# Autodesk Inventor assembly: Full_Design
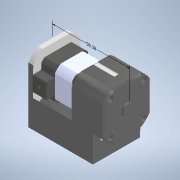
[picture p0: Inventor's stored thumbnail of the model, 180x180]
Saved by Autodesk Inventor 2022 (Build 260153000, 153)
## iProperties
Created: 2022-02-10
Part Number: Full_Design
Document SubType Name: Assembly
Designer: Mlees
Author: Mlees
## Documents named in this file (12)
- C:\Users\Mlees\Desktop\504Engineering\Stepper-Servo_Based_Robotic_Arm\Designs\Version_7\Full_Design.iam
- C:\Users\Mlees\Desktop\504Engineering\Stepper-Servo_Based_Robotic_Arm\Designs\Version_7\Downloaded_Parts\124125202-9-stp-mtr-17040w\stp-mtr-17040w.ipt
- C:\Users\Mlees\Desktop\504Engineering\Stepper-Servo_Based_Robotic_Arm\Designs\Version_7\Created_Parts\Combined_Gear_Box.ipt
- C:\Users\Mlees\Desktop\504Engineering\Stepper-Servo_Based_Robotic_Arm\Designs\Version_7\Created_Parts\Combined_Gear_Box_Modified.ipt
- C:\Users\Mlees\Desktop\504Engineering\Stepper-Servo_Based_Robotic_Arm\Designs\Version_7\Downloaded_Parts\nema17-speed-reducer-1.snapshot.9\M3 Insert 5D x 6L.step.ipt
- C:\Users\Mlees\Desktop\504Engineering\Stepper-Servo_Based_Robotic_Arm\Designs\Version_7\Downloaded_Parts\91290A101_Black-Oxide Alloy Steel Socket Head Screw_M3_6mm.ipt
- C:\Users\Mlees\Desktop\504Engineering\Stepper-Servo_Based_Robotic_Arm\Designs\Version_7\Downloaded_Parts\91290A059_Black-Oxide Alloy Steel Socket Head Screw_M3_30mm.ipt
- C:\Users\Mlees\Desktop\504Engineering\Stepper-Servo_Based_Robotic_Arm\Designs\Version_7\Created_Parts\24_Teeth_Sun_Gear.ipt
- C:\Users\Mlees\Desktop\504Engineering\Stepper-Servo_Based_Robotic_Arm\Designs\Version_7\Created_Parts\Planet_Carrier_Modifed_with_sun_gear.ipt
- C:\Users\Mlees\Desktop\504Engineering\Stepper-Servo_Based_Robotic_Arm\Designs\Version_7\Created_Parts\36_Teeth_Planet_Gear.ipt
- C:\Users\Mlees\Desktop\504Engineering\Stepper-Servo_Based_Robotic_Arm\Designs\Version_7\Created_Parts\Plamet_Carrier.ipt
- C:\Users\Mlees\Desktop\504Engineering\Stepper-Servo_Based_Robotic_Arm\Designs\Version_7\Created_Parts\Gear_Cover_modified.ipt
## Components (29 placed, 11 different names)
1. Combined_Gear_Box:1 — Rigid:1, Rigid:2, Rigid:3, Rigid:4, Rigid:7, Rigid:8, Rotational:1, Rotational:2, Rotational:3, Rotational:4, Rotational:5, Rotational:6, Rigid:9
2. Combined_Gear_Box_Modified:1 — Rigid:5, Rigid:6, Rigid:7
3. M3 Insert 5D x 6L.step:1 — Rigid:2
4. M3 Insert 5D x 6L.step:2 — Rigid:1
5. M3 Insert 5D x 6L.step:3 — Rigid:3
6. M3 Insert 5D x 6L.step:4 — Rigid:4
7. M3 Insert 5D x 6L.step:5 — Rigid:6
8. M3 Insert 5D x 6L.step:6 — Rigid:5
9. stp-mtr-17040w:1 — Rigid:8, Rotational:7, Rotational:11
10. 91290A101_Black-Oxide Alloy Steel Socket Head Screw_M3_6mm:1 — Rotational:1
11. 91290A101_Black-Oxide Alloy Steel Socket Head Screw_M3_6mm:2 — Rotational:2
12. 91290A101_Black-Oxide Alloy Steel Socket Head Screw_M3_6mm:3 — Rotational:3
13. 91290A101_Black-Oxide Alloy Steel Socket Head Screw_M3_6mm:4 — Rotational:4
14. 91290A059_Black-Oxide Alloy Steel Socket Head Screw_M3_30mm:1 — Rotational:6
15. 91290A059_Black-Oxide Alloy Steel Socket Head Screw_M3_30mm:2 — Rotational:5
16. 24_Teeth_Sun_Gear:1 — Rotational:7
17. Planet_Carrier_Modifed_with_sun_gear:1 — Rotational:8, Rotational:9, Rotational:10, Rotational:11, Rotational:15
18. 36_Teeth_Planet_Gear:1 — Rotational:9
19. 36_Teeth_Planet_Gear:2 — Rotational:8
20. 36_Teeth_Planet_Gear:3 — Rotational:10
21. 36_Teeth_Planet_Gear:4 — Rotational:12
22. 36_Teeth_Planet_Gear:5 — Rotational:13
23. 36_Teeth_Planet_Gear:6 — Rotational:14
24. Plamet_Carrier:1 — Rotational:12, Rotational:13, Rotational:14, Rotational:15
25. Gear_Cover_modified:1 — Rigid:9, Rotational:16, Rotational:17, Rotational:18, Rotational:19
26. 91290A059_Black-Oxide Alloy Steel Socket Head Screw_M3_30mm:3 — Rotational:16
27. 91290A059_Black-Oxide Alloy Steel Socket Head Screw_M3_30mm:4 — Rotational:17
28. 91290A059_Black-Oxide Alloy Steel Socket Head Screw_M3_30mm:5 — Rotational:18
29. 91290A059_Black-Oxide Alloy Steel Socket Head Screw_M3_30mm:6 — Rotational:19
## Relationships (28: RevoluteJoint 19, WeldJoint 9)
- Rigid:1 [WeldJoint]: Combined_Gear_Box:1 ↔ M3 Insert 5D x 6L.step:2
- Rigid:2 [WeldJoint]: Combined_Gear_Box:1 ↔ M3 Insert 5D x 6L.step:1
- Rigid:3 [WeldJoint]: Combined_Gear_Box:1 ↔ M3 Insert 5D x 6L.step:3
- Rigid:4 [WeldJoint]: Combined_Gear_Box:1 ↔ M3 Insert 5D x 6L.step:4
- Rigid:5 [WeldJoint]: Combined_Gear_Box_Modified:1 ↔ M3 Insert 5D x 6L.step:6
- Rigid:6 [WeldJoint]: Combined_Gear_Box_Modified:1 ↔ M3 Insert 5D x 6L.step:5
- Rigid:7 [WeldJoint]: Combined_Gear_Box:1 ↔ Combined_Gear_Box_Modified:1
- Rigid:8 [WeldJoint]: Combined_Gear_Box:1 ↔ stp-mtr-17040w:1
- Rotational:1 [RevoluteJoint]: Combined_Gear_Box:1 ↔ 91290A101_Black-Oxide Alloy Steel Socket Head Screw_M3_6mm:1
- Rotational:2 [RevoluteJoint]: Combined_Gear_Box:1 ↔ 91290A101_Black-Oxide Alloy Steel Socket Head Screw_M3_6mm:2
- Rotational:3 [RevoluteJoint]: Combined_Gear_Box:1 ↔ 91290A101_Black-Oxide Alloy Steel Socket Head Screw_M3_6mm:3
- Rotational:4 [RevoluteJoint]: Combined_Gear_Box:1 ↔ 91290A101_Black-Oxide Alloy Steel Socket Head Screw_M3_6mm:4
- Rotational:5 [RevoluteJoint]: Combined_Gear_Box:1 ↔ 91290A059_Black-Oxide Alloy Steel Socket Head Screw_M3_30mm:2
- Rotational:6 [RevoluteJoint]: Combined_Gear_Box:1 ↔ 91290A059_Black-Oxide Alloy Steel Socket Head Screw_M3_30mm:1
- Rotational:7 [RevoluteJoint]: stp-mtr-17040w:1 ↔ 24_Teeth_Sun_Gear:1
- Rotational:8 [RevoluteJoint]: Planet_Carrier_Modifed_with_sun_gear:1 ↔ 36_Teeth_Planet_Gear:2
- Rotational:9 [RevoluteJoint]: Planet_Carrier_Modifed_with_sun_gear:1 ↔ 36_Teeth_Planet_Gear:1
- Rotational:10 [RevoluteJoint]: Planet_Carrier_Modifed_with_sun_gear:1 ↔ 36_Teeth_Planet_Gear:3
- Rotational:11 [RevoluteJoint] (1 mm): stp-mtr-17040w:1 ↔ Planet_Carrier_Modifed_with_sun_gear:1
- Rotational:12 [RevoluteJoint]: 36_Teeth_Planet_Gear:4 ↔ Plamet_Carrier:1
- Rotational:13 [RevoluteJoint]: 36_Teeth_Planet_Gear:5 ↔ Plamet_Carrier:1
- Rotational:14 [RevoluteJoint]: 36_Teeth_Planet_Gear:6 ↔ Plamet_Carrier:1
- Rotational:15 [RevoluteJoint]: Planet_Carrier_Modifed_with_sun_gear:1 ↔ Plamet_Carrier:1
- Rigid:9 [WeldJoint]: Combined_Gear_Box:1 ↔ Gear_Cover_modified:1
- Rotational:16 [RevoluteJoint]: Gear_Cover_modified:1 ↔ 91290A059_Black-Oxide Alloy Steel Socket Head Screw_M3_30mm:3
- Rotational:17 [RevoluteJoint]: Gear_Cover_modified:1 ↔ 91290A059_Black-Oxide Alloy Steel Socket Head Screw_M3_30mm:4
- Rotational:18 [RevoluteJoint]: Gear_Cover_modified:1 ↔ 91290A059_Black-Oxide Alloy Steel Socket Head Screw_M3_30mm:5
- Rotational:19 [RevoluteJoint]: Gear_Cover_modified:1 ↔ 91290A059_Black-Oxide Alloy Steel Socket Head Screw_M3_30mm:6
